# Autodesk Inventor assembly: Cuvette-Sampleholder
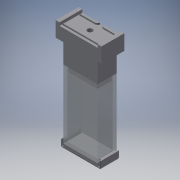
[picture p0: Inventor's stored thumbnail of the model, 180x180]
Saved by Autodesk Inventor 2016 (Build 200138000, 138)
## iProperties
Created: 2018-07-25
Part Number: Cuvette-Sampleholder
Document SubType Name: Assembly
Designer: voigt
Author: voigt
## Documents named in this file (4)
- D:\Microscope_Design\CAD_Files\Designs\mesoSPIM\Sample-Handling\Cuvette-Sampleholder\Cuvette-Sampleholder.iam
- D:\Microscope_Design\CAD_Files\Designs\mesoSPIM\Sample-Handling\Cuvette-Sampleholder\10x20mm_Cuvette_Top.ipt
- D:\Microscope_Design\CAD_Files\Library_Files\Hellma\Küvette_20mm.ipt
- D:\Microscope_Design\CAD_Files\Designs\mesoSPIM\Sample-Handling\Cuvette-Sampleholder\10x20mm_Cuvette_Bottom.ipt
## Components (3 placed, 3 different names)
1. 10x20mm_Cuvette_Top:1 — Mate:1, Flush:1, Flush:2
2. Küvette_20mm:1 — Mate:1, Flush:1, Flush:2, Flush:3
3. 10x20mm_Cuvette_Bottom:1 — Flush:3
## Relationships (4: Flush 3, Mate 1)
- Mate:1: 10x20mm_Cuvette_Top:1 ↔ Küvette_20mm:1
- Flush:1: 10x20mm_Cuvette_Top:1 ↔ Küvette_20mm:1
- Flush:2: 10x20mm_Cuvette_Top:1 ↔ Küvette_20mm:1
- Flush:3: Küvette_20mm:1 ↔ 10x20mm_Cuvette_Bottom:1
